# Autodesk Inventor assembly: Assembly9 (Crank Case Sub Assembly)
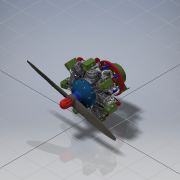
[picture p0: Inventor's stored thumbnail of the model, 180x180]
Saved by Autodesk Inventor 2018 (Build 220112000, 112)
## iProperties
Created: 2023-05-02
Part Number: Assembly9 (Crank Case Sub Assembly)
Document SubType Name: Assembly
Designer: Habib Mohamed
Author: Habib Mohamed
## Documents named in this file (25)
- D:\Inventor\My projects\Rotary Engine\Assembly\Assembly9 (Crank Case Sub Assembly).iam
- D:\Inventor\My projects\Rotary Engine\Main Block (Crank Case).ipt
- D:\Inventor\My projects\Rotary Engine\Assembly\Assembly8 (Cylinder Complete Sub Assembly).iam
- D:\Inventor\My projects\Rotary Engine\Assembly\Assembly6(Piston Sub Assembly Major).iam
- C:\Users\Habib Mohamed\Documents\Inventor\Content Center Files\R2018\en-US\ISO 4762(1)\DIN EN ISO 4762 - M4 x 12.ipt
- D:\Inventor\My projects\Rotary Engine\Assembly\Assembly10(Suction houe sub assembly).iam
- D:\Inventor\My projects\Rotary Engine\Component 9 (Suspension Spacer).ipt
- D:\Inventor\My projects\Rotary Engine\Component 10(Assembly Ring).ipt
- D:\Inventor\My projects\Rotary Engine\Assembly\Exhaust Pipe Sub-Assembly.iam
- D:\Inventor\My projects\Rotary Engine\Assembly\Assembly2 (Intake Pipe Sub Assembly).iam
- D:\Inventor\My projects\Rotary Engine\Component 46(Engine Gas Collector).ipt
- C:\Users\Habib Mohamed\Documents\Inventor\Content Center Files\R2018\en-US\ISO 4762(1)\DIN EN ISO 4762 - M3 x 5.ipt
- C:\Users\Habib Mohamed\Documents\Inventor\Content Center Files\R2018\en-US\ISO 4762(1)\DIN EN ISO 4762 - M4 x 8.ipt
- C:\Users\Habib Mohamed\Documents\Inventor\Content Center Files\R2018\en-US\ISO 10511\ISO 10511 - M5.ipt
- D:\Inventor\My projects\Rotary Engine\Assembly\Assembly11 (Cam Sub Assembly).iam
- D:\Inventor\My projects\Rotary Engine\Component 20 (Planet Wheel).ipt
- D:\Inventor\My projects\Rotary Engine\Component 3 (Planet Gear Axis).ipt
- C:\Users\Habib Mohamed\Documents\Inventor\Content Center Files\R2018\en-US\DIN 618 - T1  HK\DIN 618 - HK0609 - 6 x 10 x 9.ipt
- C:\Users\Habib Mohamed\Documents\Inventor\Content Center Files\R2018\en-US\DIN 6799\DIN 6799 - 6 7.ipt
- D:\Inventor\My projects\Rotary Engine\Assembly\Assembly13 (Cam hosuing sub ).iam
- C:\Users\Habib Mohamed\Documents\Inventor\Content Center Files\R2018\en-US\ISO 4762(1)\DIN EN ISO 4762 - M4 x 30.ipt
- D:\Inventor\My projects\Rotary Engine\Component 43(Engine Cone).ipt
- D:\Inventor\My projects\Rotary Engine\Component 42(Minehmer).ipt
- D:\Inventor\My projects\Rotary Engine\Component 44(Engine Nose).ipt
- D:\Inventor\My projects\Rotary Engine\Component 53(Propeller).ipt
## Components (128 placed, 24 different names)
1. Main Block (Crank Case):1 — Mate:1, Mate:2, Mate:3, Mate:4, Mate:6, Mate:7, Mate:8, Mate:9, Mate:10, Mate:11, Mate:12, Mate:13, Mate:14, Mate:16, Mate:18, Mate:20, Mate:22, Mate:23, Mate:24, Mate:25, Mate:26, Mate:27, Mate:28, Mate:37, Mate:48, Mate:50, Mate:52, Mate:54, Mate:56, Mate:58, Mate:60, Mate:65, Mate:66, Mate:67, Mate:68, Mate:69, Mate:70, Mate:74, Mate:75, Mate:76, Mate:90, Mate:92, Mate:93, Mate:98, Mate:100, Mate:102, Mate:104, Mate:106, Mate:108, Mate:110
2. Assembly6(Piston Sub Assembly Major):1 [sub-assembly] — Mate:1, Mate:5, Mate:6, Mate:7, Mate:8, Mate:9, Mate:10, Mate:11, Mate:12, Mate:89, Mate:91, Mate:112, Mate:113, Mate:114, Mate:115, Mate:117, Mate:119
3. Assembly10(Suction houe sub assembly):1 [sub-assembly] — Mate:23, Mate:24, Mate:25, Mate:49, Mate:51, Mate:53, Mate:55, Mate:57, Mate:59, Mate:61
4. Component 10(Assembly Ring):1 — Mate:28, Mate:29, Mate:30, Mate:63
5. Component 46(Engine Gas Collector):1 — Mate:37, Mate:38, Mate:39, Mate:64
6. DIN EN ISO 4762 M4 x 8:1 — Mate:48, Mate:49
7. DIN EN ISO 4762 M4 x 8:2 — Mate:50, Mate:51
8. DIN EN ISO 4762 M4 x 8:3 — Mate:52, Mate:53
9. DIN EN ISO 4762 M4 x 8:4 — Mate:54, Mate:55
10. DIN EN ISO 4762 M4 x 8:5 — Mate:56, Mate:57
11. DIN EN ISO 4762 M4 x 8:6 — Mate:58, Mate:59
12. DIN EN ISO 4762 M4 x 8:7 — Mate:60, Mate:61
13. Assembly11 (Cam Sub Assembly):1 [sub-assembly] — Mate:89, Mate:90, Tangent:1, Tangent:2
14. Component 20 (Planet Wheel):1 — Mate:72, Mate:76
15. Component 20 (Planet Wheel):2 — Mate:73, Mate:74
16. Component 20 (Planet Wheel):3 — Mate:71, Mate:75
17. Component 3 (Planet Gear Axis):1 — Mate:65, Mate:68, Mate:71, Mate:79, Mate:80, Mate:85
18. Component 3 (Planet Gear Axis):2 — Mate:67, Mate:70, Mate:72, Mate:77, Mate:78, Mate:87
19. Component 3 (Planet Gear Axis):3 — Mate:66, Mate:69, Mate:73, Mate:81, Mate:82, Mate:83
20. DIN 618 - T1 HK HK0609 - 6 x 10 x 9:1 — Mate:77, Mate:78, Mate:88
21. DIN 618 - T1 HK HK0609 - 6 x 10 x 9:2 — Mate:79, Mate:80, Mate:86
22. DIN 618 - T1 HK HK0609 - 6 x 10 x 9:3 — Mate:81, Mate:82, Mate:84
23. DIN 6799 6:1 — Mate:83, Mate:84
24. DIN 6799 6:2 — Mate:85, Mate:86
25. DIN 6799 6:3 — Mate:87, Mate:88
26. Assembly13 (Cam hosuing sub ):1 [sub-assembly] — Mate:91, Mate:92, Mate:93, Mate:94, Mate:95, Mate:96, Mate:97, Mate:99, Mate:101, Mate:103, Mate:105, Mate:107, Mate:109, Mate:111, Mate:116
27. DIN EN ISO 4762 M4 x 30:1 — Mate:98, Mate:99
28. DIN EN ISO 4762 M4 x 30:2 — Mate:100, Mate:101
29. DIN EN ISO 4762 M4 x 30:3 — Mate:102, Mate:103
30. DIN EN ISO 4762 M4 x 30:4 — Mate:104, Mate:105
31. DIN EN ISO 4762 M4 x 30:5 — Mate:106, Mate:107
32. DIN EN ISO 4762 M4 x 30:6 — Mate:108, Mate:109
33. DIN EN ISO 4762 M4 x 30:7 — Mate:110, Mate:111
34. Component 43(Engine Cone):1 — Mate:112, Mate:113, Mate:114
35. Component 42(Minehmer):1 — Mate:115, Mate:116, Mate:118
36. Component 44(Engine Nose):1 — Mate:119, Mate:120
37. Component 53(Propeller):1 — Mate:117, Mate:118, Mate:120
38. Assembly8 (Cylinder Complete Sub Assembly):1 [sub-assembly] — Mate:2, Mate:3, Mate:4, Mate:5, Mate:13, Mate:15, Mate:17, Mate:19, Mate:21, Mate:94, Mate:95, Mate:96, Mate:97
39. DIN EN ISO 4762 M4 x 12:1 — Mate:14, Mate:15
40. DIN EN ISO 4762 M4 x 12:2 — Mate:16, Mate:17
41. DIN EN ISO 4762 M4 x 12:3 — Mate:18, Mate:19
42. DIN EN ISO 4762 M4 x 12:4 — Mate:20, Mate:21
43. Assembly8 (Cylinder Complete Sub Assembly):2 [sub-assembly]
44. DIN EN ISO 4762 M4 x 12:5
45. DIN EN ISO 4762 M4 x 12:6
46. DIN EN ISO 4762 M4 x 12:7
47. DIN EN ISO 4762 M4 x 12:8
48. Assembly8 (Cylinder Complete Sub Assembly):3 [sub-assembly]
49. DIN EN ISO 4762 M4 x 12:9
50. DIN EN ISO 4762 M4 x 12:10
51. DIN EN ISO 4762 M4 x 12:11
52. DIN EN ISO 4762 M4 x 12:12
53. Assembly8 (Cylinder Complete Sub Assembly):4 [sub-assembly]
54. DIN EN ISO 4762 M4 x 12:13
55. DIN EN ISO 4762 M4 x 12:14
56. DIN EN ISO 4762 M4 x 12:15
57. DIN EN ISO 4762 M4 x 12:16
58. Assembly8 (Cylinder Complete Sub Assembly):5 [sub-assembly] — Mate:31, Mate:32, Mate:33, Mate:34, Mate:35, Mate:36, Mate:40, Mate:42, Mate:44, Mate:46, Tangent:1, Tangent:2
59. DIN EN ISO 4762 M4 x 12:17
60. DIN EN ISO 4762 M4 x 12:18
61. DIN EN ISO 4762 M4 x 12:19
62. DIN EN ISO 4762 M4 x 12:20
63. Assembly8 (Cylinder Complete Sub Assembly):6 [sub-assembly]
64. DIN EN ISO 4762 M4 x 12:21
65. DIN EN ISO 4762 M4 x 12:22
66. DIN EN ISO 4762 M4 x 12:23
67. DIN EN ISO 4762 M4 x 12:24
68. Assembly8 (Cylinder Complete Sub Assembly):7 [sub-assembly]
69. DIN EN ISO 4762 M4 x 12:25
70. DIN EN ISO 4762 M4 x 12:26
71. DIN EN ISO 4762 M4 x 12:27
72. DIN EN ISO 4762 M4 x 12:28
73. DIN EN ISO 4762 M3 x 5:2 — Mate:42, Mate:43
74. DIN EN ISO 4762 M3 x 5:1 — Mate:40, Mate:41
75. Assembly2 (Intake Pipe Sub Assembly):1 [sub-assembly] — Mate:31, Mate:32, Mate:33, Mate:41, Mate:43
76. Exhaust Pipe Sub-Assembly:1 [sub-assembly] — Mate:34, Mate:35, Mate:36, Mate:38, Mate:39, Mate:45, Mate:47
77. DIN EN ISO 4762 M3 x 5:3 — Mate:44, Mate:45
78. DIN EN ISO 4762 M3 x 5:4 — Mate:46, Mate:47
79. Component 9 (Suspension Spacer):1 — Mate:26, Mate:27, Mate:29, Mate:30, Mate:62
80. DIN EN ISO 10511 M5:1 — Mate:62, Mate:63
81. DIN EN ISO 4762 M3 x 5:5
82. DIN EN ISO 4762 M3 x 5:6
83. Assembly2 (Intake Pipe Sub Assembly):2 [sub-assembly]
84. Exhaust Pipe Sub-Assembly:2 [sub-assembly]
85. DIN EN ISO 4762 M3 x 5:7
86. DIN EN ISO 4762 M3 x 5:8
87. Component 9 (Suspension Spacer):2
88. DIN EN ISO 10511 M5:2
89. DIN EN ISO 4762 M3 x 5:9
90. DIN EN ISO 4762 M3 x 5:10
91. Assembly2 (Intake Pipe Sub Assembly):3 [sub-assembly]
92. Exhaust Pipe Sub-Assembly:3 [sub-assembly]
93. DIN EN ISO 4762 M3 x 5:11
94. DIN EN ISO 4762 M3 x 5:12
95. Component 9 (Suspension Spacer):3
96. DIN EN ISO 10511 M5:3
97. DIN EN ISO 4762 M3 x 5:13
98. DIN EN ISO 4762 M3 x 5:14
99. Assembly2 (Intake Pipe Sub Assembly):4 [sub-assembly]
100. Exhaust Pipe Sub-Assembly:4 [sub-assembly]
101. DIN EN ISO 4762 M3 x 5:15
102. DIN EN ISO 4762 M3 x 5:16
103. Component 9 (Suspension Spacer):4
104. DIN EN ISO 10511 M5:4
105. DIN EN ISO 4762 M3 x 5:17
106. DIN EN ISO 4762 M3 x 5:18
107. Assembly2 (Intake Pipe Sub Assembly):5 [sub-assembly]
108. Exhaust Pipe Sub-Assembly:5 [sub-assembly]
109. DIN EN ISO 4762 M3 x 5:19
110. DIN EN ISO 4762 M3 x 5:20
111. Component 9 (Suspension Spacer):5
112. DIN EN ISO 10511 M5:5
113. DIN EN ISO 4762 M3 x 5:21
114. DIN EN ISO 4762 M3 x 5:22
115. Assembly2 (Intake Pipe Sub Assembly):6 [sub-assembly]
116. Exhaust Pipe Sub-Assembly:6 [sub-assembly]
117. DIN EN ISO 4762 M3 x 5:23
118. DIN EN ISO 4762 M3 x 5:24
119. Component 9 (Suspension Spacer):6
120. DIN EN ISO 10511 M5:6
121. DIN EN ISO 4762 M3 x 5:25
122. DIN EN ISO 4762 M3 x 5:26
123. Assembly2 (Intake Pipe Sub Assembly):7 [sub-assembly]
124. Exhaust Pipe Sub-Assembly:7 [sub-assembly]
125. DIN EN ISO 4762 M3 x 5:27
126. DIN EN ISO 4762 M3 x 5:28
127. Component 9 (Suspension Spacer):7
128. DIN EN ISO 10511 M5:7
## Component patterns: (7 elements, first: Assembly8 (Cylinder Complete Sub Assembly):1 + DIN EN ISO 4762 M4 x 12:1 + DIN EN ISO 4762 M4 x 12:2 + DIN EN ISO 4762 M4 x 12:3 + DIN EN ISO 4762 M4 x 12:4), (7 elements, first: DIN EN ISO 4762 M3 x 5:2 + DIN EN ISO 4762 M3 x 5:1 + Assembly2 (Intake Pipe Sub Assembly):1 + Exhaust Pipe Sub-Assembly:1 + DIN EN ISO 4762 M3 x 5:3 + DIN EN ISO 4762 M3 x 5:4 + Component 9 (Suspension Spacer):1 + DIN EN ISO 10511 M5:1)
## Relationships (122: Mate 120, Tangent 2)
- Mate:1: Main Block (Crank Case):1 ↔ Assembly6(Piston Sub Assembly Major):1
- Mate:2: Main Block (Crank Case):1 ↔ Assembly8 (Cylinder Complete Sub Assembly):1
- Mate:3: Main Block (Crank Case):1 ↔ Assembly8 (Cylinder Complete Sub Assembly):1
- Mate:4: Main Block (Crank Case):1 ↔ Assembly8 (Cylinder Complete Sub Assembly):1
- Mate:5: Assembly6(Piston Sub Assembly Major):1 ↔ Assembly8 (Cylinder Complete Sub Assembly):1
- Mate:6: Main Block (Crank Case):1 ↔ Assembly6(Piston Sub Assembly Major):1
- Mate:7: Main Block (Crank Case):1 ↔ Assembly6(Piston Sub Assembly Major):1
- Mate:8: Main Block (Crank Case):1 ↔ Assembly6(Piston Sub Assembly Major):1
- Mate:9: Main Block (Crank Case):1 ↔ Assembly6(Piston Sub Assembly Major):1
- Mate:10: Main Block (Crank Case):1 ↔ Assembly6(Piston Sub Assembly Major):1
- Mate:11: Main Block (Crank Case):1 ↔ Assembly6(Piston Sub Assembly Major):1
- Mate:12: Main Block (Crank Case):1 ↔ Assembly6(Piston Sub Assembly Major):1
- Mate:13: Main Block (Crank Case):1 ↔ Assembly8 (Cylinder Complete Sub Assembly):1
- Mate:14: Main Block (Crank Case):1 ↔ DIN EN ISO 4762 M4 x 12:1
- Mate:15: Assembly8 (Cylinder Complete Sub Assembly):1 ↔ DIN EN ISO 4762 M4 x 12:1
- Mate:16: Main Block (Crank Case):1 ↔ DIN EN ISO 4762 M4 x 12:2
- Mate:17: Assembly8 (Cylinder Complete Sub Assembly):1 ↔ DIN EN ISO 4762 M4 x 12:2
- Mate:18: Main Block (Crank Case):1 ↔ DIN EN ISO 4762 M4 x 12:3
- Mate:19: Assembly8 (Cylinder Complete Sub Assembly):1 ↔ DIN EN ISO 4762 M4 x 12:3
- Mate:20: Main Block (Crank Case):1 ↔ DIN EN ISO 4762 M4 x 12:4
- Mate:21: Assembly8 (Cylinder Complete Sub Assembly):1 ↔ DIN EN ISO 4762 M4 x 12:4
- Mate:22: Main Block (Crank Case):1
- Mate:23: Main Block (Crank Case):1 ↔ Assembly10(Suction houe sub assembly):1
- Mate:24: Main Block (Crank Case):1 ↔ Assembly10(Suction houe sub assembly):1
- Mate:25: Main Block (Crank Case):1 ↔ Assembly10(Suction houe sub assembly):1
- Mate:26: Main Block (Crank Case):1 ↔ Component 9 (Suspension Spacer):1
- Mate:27: Main Block (Crank Case):1 ↔ Component 9 (Suspension Spacer):1
- Mate:28: Main Block (Crank Case):1 ↔ Component 10(Assembly Ring):1
- Mate:29: Component 10(Assembly Ring):1 ↔ Component 9 (Suspension Spacer):1
- Mate:30: Component 10(Assembly Ring):1 ↔ Component 9 (Suspension Spacer):1
- Mate:31: Assembly8 (Cylinder Complete Sub Assembly):5 ↔ Assembly2 (Intake Pipe Sub Assembly):1
- Mate:32: Assembly8 (Cylinder Complete Sub Assembly):5 ↔ Assembly2 (Intake Pipe Sub Assembly):1
- Mate:33: Assembly8 (Cylinder Complete Sub Assembly):5 ↔ Assembly2 (Intake Pipe Sub Assembly):1
- Mate:34: Assembly8 (Cylinder Complete Sub Assembly):5 ↔ Exhaust Pipe Sub-Assembly:1
- Mate:35: Assembly8 (Cylinder Complete Sub Assembly):5 ↔ Exhaust Pipe Sub-Assembly:1
- Mate:36: Assembly8 (Cylinder Complete Sub Assembly):5 ↔ Exhaust Pipe Sub-Assembly:1
- Mate:37: Main Block (Crank Case):1 ↔ Component 46(Engine Gas Collector):1
- Mate:38: Component 46(Engine Gas Collector):1 ↔ Exhaust Pipe Sub-Assembly:1
- Mate:39: Component 46(Engine Gas Collector):1 ↔ Exhaust Pipe Sub-Assembly:1
- Mate:40: Assembly8 (Cylinder Complete Sub Assembly):5 ↔ DIN EN ISO 4762 M3 x 5:1
- Mate:41: DIN EN ISO 4762 M3 x 5:1 ↔ Assembly2 (Intake Pipe Sub Assembly):1
- Mate:42: Assembly8 (Cylinder Complete Sub Assembly):5 ↔ DIN EN ISO 4762 M3 x 5:2
- Mate:43: DIN EN ISO 4762 M3 x 5:2 ↔ Assembly2 (Intake Pipe Sub Assembly):1
- Mate:44: Assembly8 (Cylinder Complete Sub Assembly):5 ↔ DIN EN ISO 4762 M3 x 5:3
- Mate:45: Exhaust Pipe Sub-Assembly:1 ↔ DIN EN ISO 4762 M3 x 5:3
- Mate:46: Assembly8 (Cylinder Complete Sub Assembly):5 ↔ DIN EN ISO 4762 M3 x 5:4
- Mate:47: Exhaust Pipe Sub-Assembly:1 ↔ DIN EN ISO 4762 M3 x 5:4
- Mate:48: Main Block (Crank Case):1 ↔ DIN EN ISO 4762 M4 x 8:1
- Mate:49: Assembly10(Suction houe sub assembly):1 ↔ DIN EN ISO 4762 M4 x 8:1
- Mate:50: Main Block (Crank Case):1 ↔ DIN EN ISO 4762 M4 x 8:2
- Mate:51: Assembly10(Suction houe sub assembly):1 ↔ DIN EN ISO 4762 M4 x 8:2
- Mate:52: Main Block (Crank Case):1 ↔ DIN EN ISO 4762 M4 x 8:3
- Mate:53: Assembly10(Suction houe sub assembly):1 ↔ DIN EN ISO 4762 M4 x 8:3
- Mate:54: Main Block (Crank Case):1 ↔ DIN EN ISO 4762 M4 x 8:4
- Mate:55: Assembly10(Suction houe sub assembly):1 ↔ DIN EN ISO 4762 M4 x 8:4
- Mate:56: Main Block (Crank Case):1 ↔ DIN EN ISO 4762 M4 x 8:5
- Mate:57: Assembly10(Suction houe sub assembly):1 ↔ DIN EN ISO 4762 M4 x 8:5
- Mate:58: Main Block (Crank Case):1 ↔ DIN EN ISO 4762 M4 x 8:6
- Mate:59: Assembly10(Suction houe sub assembly):1 ↔ DIN EN ISO 4762 M4 x 8:6
- Mate:60: Main Block (Crank Case):1 ↔ DIN EN ISO 4762 M4 x 8:7
- Mate:61: Assembly10(Suction houe sub assembly):1 ↔ DIN EN ISO 4762 M4 x 8:7
- Mate:62: Component 9 (Suspension Spacer):1 ↔ DIN EN ISO 10511 M5:1
- Mate:63: Component 10(Assembly Ring):1 ↔ DIN EN ISO 10511 M5:1
- Mate:64: Component 46(Engine Gas Collector):1
- Mate:65: Main Block (Crank Case):1 ↔ Component 3 (Planet Gear Axis):1
- Mate:66: Main Block (Crank Case):1 ↔ Component 3 (Planet Gear Axis):3
- Mate:67: Main Block (Crank Case):1 ↔ Component 3 (Planet Gear Axis):2
- Mate:68: Main Block (Crank Case):1 ↔ Component 3 (Planet Gear Axis):1
- Mate:69: Main Block (Crank Case):1 ↔ Component 3 (Planet Gear Axis):3
- Mate:70: Main Block (Crank Case):1 ↔ Component 3 (Planet Gear Axis):2
- Mate:71: Component 20 (Planet Wheel):3 ↔ Component 3 (Planet Gear Axis):1
- Mate:72: Component 20 (Planet Wheel):1 ↔ Component 3 (Planet Gear Axis):2
- Mate:73: Component 20 (Planet Wheel):2 ↔ Component 3 (Planet Gear Axis):3
- Mate:74: Main Block (Crank Case):1 ↔ Component 20 (Planet Wheel):2
- Mate:75: Main Block (Crank Case):1 ↔ Component 20 (Planet Wheel):3
- Mate:76: Main Block (Crank Case):1 ↔ Component 20 (Planet Wheel):1
- Mate:77: Component 3 (Planet Gear Axis):2 ↔ DIN 618 - T1 HK HK0609 - 6 x 10 x 9:1
- Mate:78: Component 3 (Planet Gear Axis):2 ↔ DIN 618 - T1 HK HK0609 - 6 x 10 x 9:1
- Mate:79: Component 3 (Planet Gear Axis):1 ↔ DIN 618 - T1 HK HK0609 - 6 x 10 x 9:2
- Mate:80: Component 3 (Planet Gear Axis):1 ↔ DIN 618 - T1 HK HK0609 - 6 x 10 x 9:2
- Mate:81: Component 3 (Planet Gear Axis):3 ↔ DIN 618 - T1 HK HK0609 - 6 x 10 x 9:3
- Mate:82: Component 3 (Planet Gear Axis):3 ↔ DIN 618 - T1 HK HK0609 - 6 x 10 x 9:3
- Mate:83: Component 3 (Planet Gear Axis):3 ↔ DIN 6799 6:1
- Mate:84: DIN 618 - T1 HK HK0609 - 6 x 10 x 9:3 ↔ DIN 6799 6:1
- Mate:85: Component 3 (Planet Gear Axis):1 ↔ DIN 6799 6:2
- Mate:86: DIN 618 - T1 HK HK0609 - 6 x 10 x 9:2 ↔ DIN 6799 6:2
- Mate:87: Component 3 (Planet Gear Axis):2 ↔ DIN 6799 6:3
- Mate:88: DIN 618 - T1 HK HK0609 - 6 x 10 x 9:1 ↔ DIN 6799 6:3
- Mate:89: Assembly6(Piston Sub Assembly Major):1 ↔ Assembly11 (Cam Sub Assembly):1
- Mate:90: Main Block (Crank Case):1 ↔ Assembly11 (Cam Sub Assembly):1
- Tangent:1: Assembly11 (Cam Sub Assembly):1 ↔ Assembly8 (Cylinder Complete Sub Assembly):5
- Tangent:2: Assembly11 (Cam Sub Assembly):1 ↔ Assembly8 (Cylinder Complete Sub Assembly):5
- Mate:91: Assembly6(Piston Sub Assembly Major):1 ↔ Assembly13 (Cam hosuing sub ):1
- Mate:92: Main Block (Crank Case):1 ↔ Assembly13 (Cam hosuing sub ):1
- Mate:93: Main Block (Crank Case):1 ↔ Assembly13 (Cam hosuing sub ):1
- Mate:94: Assembly13 (Cam hosuing sub ):1 ↔ Assembly8 (Cylinder Complete Sub Assembly):1
- Mate:95: Assembly13 (Cam hosuing sub ):1 ↔ Assembly8 (Cylinder Complete Sub Assembly):1
- Mate:96: Assembly13 (Cam hosuing sub ):1 ↔ Assembly8 (Cylinder Complete Sub Assembly):1
- Mate:97: Assembly13 (Cam hosuing sub ):1 ↔ Assembly8 (Cylinder Complete Sub Assembly):1
- Mate:98: Main Block (Crank Case):1 ↔ DIN EN ISO 4762 M4 x 30:1
- Mate:99: Assembly13 (Cam hosuing sub ):1 ↔ DIN EN ISO 4762 M4 x 30:1
- Mate:100: Main Block (Crank Case):1 ↔ DIN EN ISO 4762 M4 x 30:2
- Mate:101: Assembly13 (Cam hosuing sub ):1 ↔ DIN EN ISO 4762 M4 x 30:2
- Mate:102: Main Block (Crank Case):1 ↔ DIN EN ISO 4762 M4 x 30:3
- Mate:103: Assembly13 (Cam hosuing sub ):1 ↔ DIN EN ISO 4762 M4 x 30:3
- Mate:104: Main Block (Crank Case):1 ↔ DIN EN ISO 4762 M4 x 30:4
- Mate:105: Assembly13 (Cam hosuing sub ):1 ↔ DIN EN ISO 4762 M4 x 30:4
- Mate:106: Main Block (Crank Case):1 ↔ DIN EN ISO 4762 M4 x 30:5
- Mate:107: Assembly13 (Cam hosuing sub ):1 ↔ DIN EN ISO 4762 M4 x 30:5
- Mate:108: Main Block (Crank Case):1 ↔ DIN EN ISO 4762 M4 x 30:6
- Mate:109: Assembly13 (Cam hosuing sub ):1 ↔ DIN EN ISO 4762 M4 x 30:6
- Mate:110: Main Block (Crank Case):1 ↔ DIN EN ISO 4762 M4 x 30:7
- Mate:111: Assembly13 (Cam hosuing sub ):1 ↔ DIN EN ISO 4762 M4 x 30:7
- Mate:112: Assembly6(Piston Sub Assembly Major):1 ↔ Component 43(Engine Cone):1
- Mate:113: Assembly6(Piston Sub Assembly Major):1 ↔ Component 43(Engine Cone):1
- Mate:114: Assembly6(Piston Sub Assembly Major):1 ↔ Component 43(Engine Cone):1
- Mate:115: Assembly6(Piston Sub Assembly Major):1 ↔ Component 42(Minehmer):1
- Mate:116: Assembly13 (Cam hosuing sub ):1 ↔ Component 42(Minehmer):1
- Mate:117: Assembly6(Piston Sub Assembly Major):1 ↔ Component 53(Propeller):1
- Mate:118: Component 42(Minehmer):1 ↔ Component 53(Propeller):1
- Mate:119: Assembly6(Piston Sub Assembly Major):1 ↔ Component 44(Engine Nose):1
- Mate:120: Component 44(Engine Nose):1 ↔ Component 53(Propeller):1
